# Autodesk Inventor assembly: reifen_achse
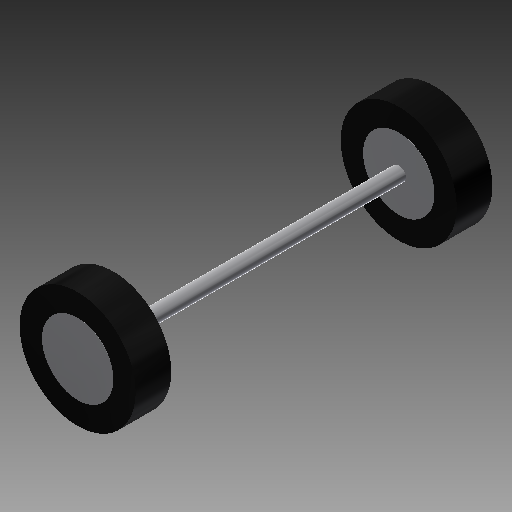
[picture p0: Inventor's stored thumbnail of the model, 512x512]
Saved by Autodesk Inventor 2018 (Build 220112000, 112)
## iProperties
Created: 2020-03-17
Part Number: reifen_achse
Material: Generisch
Document SubType Name: Assembly
Designer: wepet
Author: wepet
## Documents named in this file (4)
- C:\Users\wepet\Downloads\anhaenger\current\details\reifen\reifen_achse.iam
- C:\Users\wepet\Downloads\anhaenger\current\details\reifen\details\reifen_achse.ipt
- C:\Users\wepet\Downloads\anhaenger\current\details\reifen\details\reifen_felge.ipt
- C:\Users\wepet\Downloads\anhaenger\current\details\reifen\details\reifen_mantel.ipt
## Components (5 placed, 3 different names)
1. reifen_achse:1 — Einfügen:1, Einfügen:3
2. reifen_felge:1 — Einfügen:1, Einfügen:2
3. reifen_mantel:1 — Einfügen:2
4. reifen_felge:2 — Einfügen:3, Einfügen:4
5. reifen_mantel:2 — Einfügen:4
## Relationships (4: Insert 4)
- Einfügen:1 [Insert]: reifen_achse:1 ↔ reifen_felge:1
- Einfügen:2 [Insert]: reifen_felge:1 ↔ reifen_mantel:1
- Einfügen:3 [Insert]: reifen_achse:1 ↔ reifen_felge:2
- Einfügen:4 [Insert]: reifen_felge:2 ↔ reifen_mantel:2
